# Autodesk Inventor assembly: Telescope
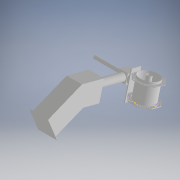
[picture p0: Inventor's stored thumbnail of the model, 180x180]
Saved by Autodesk Inventor 2022 (Build 260153000, 153)
## iProperties
RuleStatus: InUse
Created: 2021-05-06
Part Number: Telescope
Document SubType Name: Assembly
Designer: Mick Veldhuis
Author: Mick Veldhuis
## Documents named in this file (11)
- C:\Users\Mick Veldhuis\Desktop\bsc-project\inventor\observatory\Telescope.iam
- C:\Users\Mick Veldhuis\Desktop\bsc-project\inventor\observatory\MountBase.ipt
- C:\Users\Mick Veldhuis\Desktop\bsc-project\inventor\observatory\RaAxis.ipt
- C:\Users\Mick Veldhuis\Desktop\bsc-project\inventor\observatory\RaDecConnector.ipt
- C:\Users\Mick Veldhuis\Desktop\bsc-project\inventor\observatory\DecAxis.ipt
- C:\Users\Mick Veldhuis\Desktop\bsc-project\inventor\observatory\MainMirror.ipt
- PrimaryMirror.ipt
- C:\Users\Mick Veldhuis\Desktop\bsc-project\inventor\observatory\TelescopeMountConnector.ipt
- C:\Users\Mick Veldhuis\Documents\Inventor\Content Center Files\R2022\en-US\ISO 7089\ISO 7089 - 8 - 140 HV(1).ipt
- C:\Users\Mick Veldhuis\Documents\Inventor\Content Center Files\R2022\en-US\ISO 4017(1)\ISO 4017 - M8 x 35 - ISO.ipt
- C:\Users\Mick Veldhuis\Desktop\bsc-project\inventor\observatory\StrutConnector.ipt
## Components (18 placed, 9 different names)
1. MountBase:1 — RaAxisRotation
2. RaAxis:1 — RaAxisRotation, Insert:1, Insert:2
3. RaDecConnector:1 — Insert:1, Insert:2, DecAxisRotation
4. DecAxis:1 — Insert:5, Insert:6, Mate:1, Mate:2, Mate:3, Mate:4, Mate:5, Mate:6, Mate:7, Mate:8, DecAxisRotation
5. PrimaryMirror:1 — Insert:3, Insert:4, Insert:11, Insert:12, Insert:14, Insert:15, Insert:16, Insert:17, Insert:18, Insert:19
6. TelescopeMountConnector:1 — Insert:4, Insert:6, Insert:18
7. TelescopeMountConnector:2 — Insert:3, Insert:5, Insert:19
8. ISO 7089 8:1 — Mate:1, Mate:2, Insert:7
9. ISO 4017 M8 x 35:1 — Insert:7
10. ISO 7089 8:2 — Mate:3, Mate:4, Insert:8
11. ISO 4017 M8 x 35:2 — Insert:8
12. ISO 7089 8:3 — Mate:5, Mate:6, Insert:9
13. ISO 4017 M8 x 35:3 — Insert:9
14. ISO 7089 8:4 — Mate:7, Mate:8, Insert:10
15. ISO 4017 M8 x 35:4 — Insert:10
16. StrutConnector:1 — Insert:11, Insert:12
17. StrutConnector:2 — Insert:14, Insert:15
18. StrutConnector:3 — Insert:16, Insert:17
## Relationships (28: Insert 18, Mate 8, RevoluteJoint 2)
- RaAxisRotation [RevoluteJoint]: MountBase:1 ↔ RaAxis:1
- Insert:1: RaAxis:1 ↔ RaDecConnector:1
- Insert:2: RaAxis:1 ↔ RaDecConnector:1
- Insert:3: PrimaryMirror:1 ↔ TelescopeMountConnector:2
- Insert:4: PrimaryMirror:1 ↔ TelescopeMountConnector:1
- Insert:5: DecAxis:1 ↔ TelescopeMountConnector:2
- Insert:6: DecAxis:1 ↔ TelescopeMountConnector:1
- Mate:1: DecAxis:1 ↔ ISO 7089 8:1
- Mate:2: DecAxis:1 ↔ ISO 7089 8:1
- Insert:7: ISO 7089 8:1 ↔ ISO 4017 M8 x 35:1
- Mate:3: DecAxis:1 ↔ ISO 7089 8:2
- Mate:4: DecAxis:1 ↔ ISO 7089 8:2
- Insert:8: ISO 7089 8:2 ↔ ISO 4017 M8 x 35:2
- Mate:5: DecAxis:1 ↔ ISO 7089 8:3
- Mate:6: DecAxis:1 ↔ ISO 7089 8:3
- Insert:9: ISO 7089 8:3 ↔ ISO 4017 M8 x 35:3
- Mate:7: DecAxis:1 ↔ ISO 7089 8:4
- Mate:8: DecAxis:1 ↔ ISO 7089 8:4
- Insert:10: ISO 7089 8:4 ↔ ISO 4017 M8 x 35:4
- DecAxisRotation [RevoluteJoint]: RaDecConnector:1 ↔ DecAxis:1
- Insert:11: PrimaryMirror:1 ↔ StrutConnector:1
- Insert:12: PrimaryMirror:1 ↔ StrutConnector:1
- Insert:14: PrimaryMirror:1 ↔ StrutConnector:2
- Insert:15: PrimaryMirror:1 ↔ StrutConnector:2
- Insert:16: PrimaryMirror:1 ↔ StrutConnector:3
- Insert:17: PrimaryMirror:1 ↔ StrutConnector:3
- Insert:18: PrimaryMirror:1 ↔ TelescopeMountConnector:1
- Insert:19: PrimaryMirror:1 ↔ TelescopeMountConnector:2
## Named parameters: RaAngle = 0 deg, DecAngle = 0 deg, iTrigger0 = 1
